# Autodesk Inventor assembly: 00_X02598_LEGOmini_CityGuy
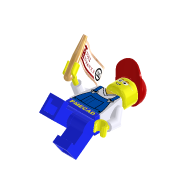
[picture p0: Inventor's stored thumbnail of the model, 180x180]
Saved by Autodesk Inventor 2022.2 (Build 262287000, 287)
## iProperties
Created: 2022-02-05
Part Number: 00_X02598_LEGOmini_CityGuy
Document SubType Name: Assembly
Designer: Jason
Author: Jason
## Documents named in this file (7)
- C:\Users\Jason\Documents\PME1017_X02598\教材_LEGOmini_20220205\00_X02598_LEGOmini_CityGuy.iam
- C:\Users\Jason\Documents\PME1017_X02598\教材_LEGOmini_20220205\X02598_LEGOmini_LowerBody.iam
- C:\Users\Jason\Documents\PME1017_X02598\教材_LEGOmini_20220205\X02598_LEGOmini_UpperBody.iam
- C:\Users\Jason\Documents\PME1017_X02598\教材_LEGOmini_20220205\X02598_LEGOmini_Head_Y.ipt
- C:\Users\Jason\Documents\PME1017_X02598\教材_LEGOmini_20220205\X02598_LEGOmini_Hat_R.ipt
- C:\Users\Jason\Documents\PME1017_X02598\教材_LEGOmini_20220205\X02598_LEGOmini_PMECAD_LEGOmini_FlagFrame.ipt
- C:\Users\Jason\Documents\PME1017_X02598\教材_LEGOmini_20220205\X02598_LEGOmini_PMECAD_LEGOmini_Flag.ipt
## Components (6 placed, 6 different names)
1. X02598_LEGOmini_LowerBody:1 [sub-assembly] — 貼合:1, 齊平:1, 齊平:2
2. X02598_LEGOmini_UpperBody:1 [sub-assembly] — 貼合:1, 齊平:1, 齊平:2, 插入:1, 插入:3
3. X02598_LEGOmini_Head_Y:1 — 插入:1, 插入:2
4. X02598_LEGOmini_Hat_R:1 — 插入:2
5. X02598_LEGOmini_PMECAD_LEGOmini_FlagFrame:1 — 插入:3, 貼合:2, 貼合:3, 相切:1
6. X02598_LEGOmini_PMECAD_LEGOmini_Flag:1 — 貼合:2, 貼合:3, 相切:1
## Relationships (9: Mate 3, Insert 3, Flush 2, Tangent 1)
- 貼合:1 [Mate]: X02598_LEGOmini_LowerBody:1 ↔ X02598_LEGOmini_UpperBody:1
- 齊平:1 [Flush]: X02598_LEGOmini_LowerBody:1 ↔ X02598_LEGOmini_UpperBody:1
- 齊平:2 [Flush]: X02598_LEGOmini_LowerBody:1 ↔ X02598_LEGOmini_UpperBody:1
- 插入:1 [Insert]: X02598_LEGOmini_UpperBody:1 ↔ X02598_LEGOmini_Head_Y:1
- 插入:2 [Insert]: X02598_LEGOmini_Head_Y:1 ↔ X02598_LEGOmini_Hat_R:1
- 插入:3 [Insert] (-3 mm): X02598_LEGOmini_UpperBody:1 ↔ X02598_LEGOmini_PMECAD_LEGOmini_FlagFrame:1
- 貼合:2 [Mate]: X02598_LEGOmini_PMECAD_LEGOmini_FlagFrame:1 ↔ X02598_LEGOmini_PMECAD_LEGOmini_Flag:1
- 貼合:3 [Mate]: X02598_LEGOmini_PMECAD_LEGOmini_FlagFrame:1 ↔ X02598_LEGOmini_PMECAD_LEGOmini_Flag:1
- 相切:1 [Tangent]: X02598_LEGOmini_PMECAD_LEGOmini_FlagFrame:1 ↔ X02598_LEGOmini_PMECAD_LEGOmini_Flag:1
